# Autodesk Inventor assembly: MG-Grundplatte
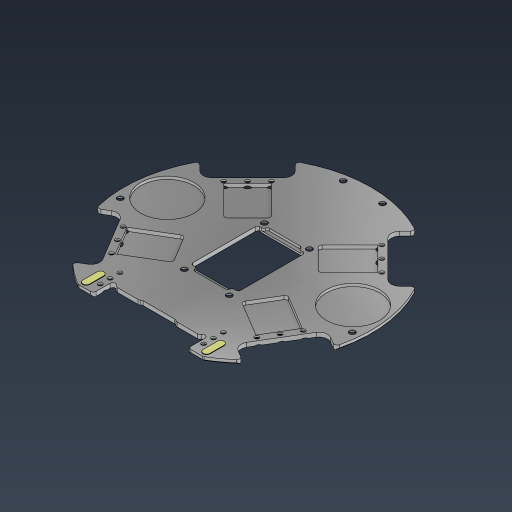
[picture p0: Inventor's stored thumbnail of the model, 512x512]
Saved by Autodesk Inventor 2023.1 (Build 271208000, 208)
## iProperties
Part Number: MG-Grundplatte
Material: Generisch
Document SubType Name: Assembly
Designer: rYan
Mass: 128.652 g
Surface Area: 395.086 cm^2
Volume: 47.6131 cm^3
Density: 2.70203 g/cm^3
Author: rYan
## Documents named in this file (3)
- D:\TIGERsGIT\Hardware\mechanik\2024\Inventor\Robot\MG-Grundplatte.iam
- D:\TIGERsGIT\Hardware\mechanik\2024\Inventor\Robot\Grundplatte.ipt
- D:\TIGERsGIT\Hardware\mechanik\2024\Inventor\Robot\Dribbler\Dribblerdaempfer Unten V2.ipt
## Components (3 placed, 2 different names)
1. Grundplatte:1 — Fluchtend:1, Passend:1, Passend:2, Passend:7, Passend:8, Passend:9, Passend:10, Tangential:3, Tangential:4
2. Dribblerdaempfer Unten V2:1 — Passend:7, Passend:10, Tangential:3
3. Dribblerdaempfer Unten V2:2 — Passend:8, Passend:9, Tangential:4
## Relationships (9: Mate 6, Tangent 2, Flush 1)
- Fluchtend:1 [Flush]: Grundplatte:1
- Passend:1 [Mate]: Grundplatte:1
- Passend:2 [Mate]: Grundplatte:1
- Passend:7 [Mate]: Grundplatte:1 ↔ Dribblerdaempfer Unten V2:1
- Passend:8 [Mate]: Grundplatte:1 ↔ Dribblerdaempfer Unten V2:2
- Passend:9 [Mate]: Grundplatte:1 ↔ Dribblerdaempfer Unten V2:2
- Passend:10 [Mate]: Grundplatte:1 ↔ Dribblerdaempfer Unten V2:1
- Tangential:3: Grundplatte:1 ↔ Dribblerdaempfer Unten V2:1
- Tangential:4: Grundplatte:1 ↔ Dribblerdaempfer Unten V2:2
